# Autodesk Inventor assembly: 372.91.330
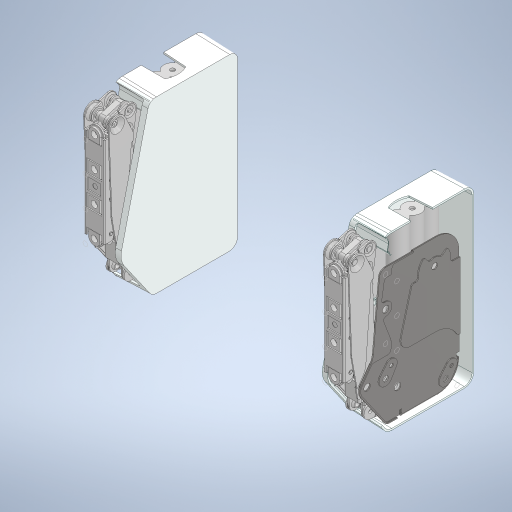
[picture p0: Inventor's stored thumbnail of the model, 512x512]
Saved by Autodesk Inventor 2024 (Build 280153000, 153)
## iProperties
RuleStatus: InUse
Created: 2019-11-19
Part Number: 372.91.330
Document SubType Name: Assembly
Designer: RokasM
Description: Hafele Free flap 3.15 107 deg mod.D
AfterDocOpen0: FrontOffset
Title: Hafele Free flap 3.15 107 deg mod.D
Revision Number: 1
## Documents named in this file (21)
- C:\W4INV 2024 Design\LIBRARY\Flap Fittings & Stays\Hafele Free flap 3.15 107 deg mod.D\Hafele_Free_flap_3.15_107_deg_mod.D.iam
- C:\W4INV 2024 Design\LIBRARY\Flap Fittings & Stays\Hafele Free flap 3.15 107 deg mod.D\Parts\372.91.410.ipt
- C:\W4INV 2024 Design\LIBRARY\Flap Fittings & Stays\Hafele Free flap 3.15 107 deg mod.D\Parts\372.91.410_1.ipt
- C:\W4INV 2024 Design\LIBRARY\Flap Fittings & Stays\Hafele Free flap 3.15 107 deg mod.D\Parts\372.91.410_2.ipt
- C:\W4INV 2024 Design\LIBRARY\Flap Fittings & Stays\Hafele Free flap 3.15 107 deg mod.D\Parts\372.91.410_3.ipt
- C:\W4INV 2024 Design\LIBRARY\Flap Fittings & Stays\Hafele Free flap 3.15 107 deg mod.D\Parts\372.91.410_4.ipt
- C:\W4INV 2024 Design\LIBRARY\Flap Fittings & Stays\Hafele Free flap 3.15 107 deg mod.D\Parts\372.91.410_5.ipt
- C:\W4INV 2024 Design\LIBRARY\Flap Fittings & Stays\Hafele Free flap 3.15 107 deg mod.D\Parts\372.91.410_6.ipt
- C:\W4INV 2024 Design\LIBRARY\Flap Fittings & Stays\Hafele Free flap 3.15 107 deg mod.D\Parts\372.91.410_7.ipt
- C:\W4INV 2024 Design\LIBRARY\Flap Fittings & Stays\Hafele Free flap 3.15 107 deg mod.D\Parts\372.91.433.ipt
- C:\W4INV 2024 Design\LIBRARY\Flap Fittings & Stays\Hafele Free flap 3.15 107 deg mod.D\Parts\372.91.410left.ipt
- C:\W4INV 2024 Design\LIBRARY\Flap Fittings & Stays\Hafele Free flap 3.15 107 deg mod.D\Parts\372.91.410_1left.ipt
- C:\W4INV 2024 Design\LIBRARY\Flap Fittings & Stays\Hafele Free flap 3.15 107 deg mod.D\Parts\372.91.410_2left.ipt
- C:\W4INV 2024 Design\LIBRARY\Flap Fittings & Stays\Hafele Free flap 3.15 107 deg mod.D\Parts\372.91.410_3left.ipt
- C:\W4INV 2024 Design\LIBRARY\Flap Fittings & Stays\Hafele Free flap 3.15 107 deg mod.D\Parts\372.91.410_4left.ipt
- C:\W4INV 2024 Design\LIBRARY\Flap Fittings & Stays\Hafele Free flap 3.15 107 deg mod.D\Parts\372.91.410_5left.ipt
- C:\W4INV 2024 Design\LIBRARY\Flap Fittings & Stays\Hafele Free flap 3.15 107 deg mod.D\Parts\372.91.410_6left.ipt
- C:\W4INV 2024 Design\LIBRARY\Flap Fittings & Stays\Hafele Free flap 3.15 107 deg mod.D\Parts\372.91.410_7left.ipt
- C:\W4INV 2024 Design\LIBRARY\Flap Fittings & Stays\Hafele Free flap 3.15 107 deg mod.D\Parts\372.91.433left.ipt
- C:\W4INV 2024 Design\LIBRARY\Flap Fittings & Stays\Hafele Free flap 3.15 107 deg mod.D\Parts\front_holes.ipt
- C:\Users\Public\Documents\Woodwork for Inventor\Textures\Black.png
## Components (20 placed, 19 different names)
1. cylinders:1 — Flush:4, Mate:4, Mate:5, Mate:6
2. door_plate:1 — Insert:5, Insert:6, Insert:7, Flush:18, Mate:20, Mate:21, Mate:22, Mate:23, Mate:27
3. upper_arm:1 — Insert:4, Insert:7, Mate:19
4. lower_arm:1 — Insert:3, Insert:6
5. swing_arm:1 — Insert:2, Insert:3
6. middle_arm:1 — Insert:1, Insert:5
7. outer_plate:1 — Flush:1, Flush:2, Flush:3, Mate:3, Flush:4, Mate:4, Mate:5, Angle:1, Flush:16, Flush:17
8. inner_plate:1 — Insert:1, Insert:2, Insert:4, Mate:1, Mate:2, Flush:2, Flush:3, Mate:3, Mate:6
9. cover:1 — Mate:1, Mate:2, Flush:1
10. cylinders_left:1 — Mate:10, Mate:11, Flush:9, Mate:12
11. door_plate_left:1 — Insert:8, Insert:9, Insert:11, Flush:18, Mate:19, Mate:20, Mate:24, Mate:25, Mate:26, Mate:28
12. upper_arm_left:1 — Insert:8, Insert:12
13. lower_arm_left:1 — Insert:9, Insert:10
14. swing_arm_left:1 — Insert:10, Insert:13
15. middle_arm_left:1 — Insert:11, Insert:14
16. outer_plate_left:1 — Mate:10, Mate:11, Flush:9, Mate:13, Flush:10, Flush:11, Flush:12, Flush:16, Flush:17
17. inner_plate_left:1 — Mate:12, Mate:13, Flush:10, Flush:11, Insert:12, Insert:13, Insert:14, Mate:14, Mate:15
18. cover_left:1 — Flush:12, Mate:14, Mate:15
19. front_holes:1 — Mate:21, Mate:22, Mate:23, Mate:27
20. front_holes:2 — Mate:24, Mate:25, Mate:26, Mate:28
## Relationships (48: Mate 22, Insert 14, Flush 11, Angle 1)
- Insert:1 (7.2 mm): middle_arm:1 ↔ inner_plate:1
- Insert:2 (2 mm): swing_arm:1 ↔ inner_plate:1
- Insert:3 (-0.55 mm): lower_arm:1 ↔ swing_arm:1
- Insert:4 (-0.3 mm): upper_arm:1 ↔ inner_plate:1
- Insert:5 (0.25 mm): door_plate:1 ↔ middle_arm:1
- Insert:6 (2.05 mm): door_plate:1 ↔ lower_arm:1
- Insert:7 (0.15 mm): door_plate:1 ↔ upper_arm:1
- Mate:1: inner_plate:1 ↔ cover:1
- Mate:2: inner_plate:1 ↔ cover:1
- Flush:1: outer_plate:1 ↔ cover:1
- Flush:2: outer_plate:1 ↔ inner_plate:1
- Flush:3: outer_plate:1 ↔ inner_plate:1
- Mate:3 (26.2 mm): outer_plate:1 ↔ inner_plate:1
- Flush:4 (-24.9 mm): cylinders:1 ↔ outer_plate:1
- Mate:4 (-14.3 mm): cylinders:1 ↔ outer_plate:1
- Mate:5 (-14.3 mm): cylinders:1 ↔ outer_plate:1
- Mate:6 (-19.92 mm): cylinders:1 ↔ inner_plate:1
- Angle:1 (0 deg): outer_plate:1
- Insert:8 (0.15 mm): door_plate_left:1 ↔ upper_arm_left:1
- Insert:9 (2.05 mm): door_plate_left:1 ↔ lower_arm_left:1
- Insert:10 (-0.55 mm): lower_arm_left:1 ↔ swing_arm_left:1
- Insert:11 (0.25 mm): door_plate_left:1 ↔ middle_arm_left:1
- Mate:10 (-14.3 mm): cylinders_left:1 ↔ outer_plate_left:1
- Mate:11 (-14.3 mm): cylinders_left:1 ↔ outer_plate_left:1
- Flush:9 (-24.9 mm): cylinders_left:1 ↔ outer_plate_left:1
- Mate:12 (-19.92 mm): cylinders_left:1 ↔ inner_plate_left:1
- Mate:13 (26.2 mm): outer_plate_left:1 ↔ inner_plate_left:1
- Flush:10: outer_plate_left:1 ↔ inner_plate_left:1
- Flush:11: outer_plate_left:1 ↔ inner_plate_left:1
- Insert:12 (-0.3 mm): upper_arm_left:1 ↔ inner_plate_left:1
- Insert:13 (2 mm): swing_arm_left:1 ↔ inner_plate_left:1
- Insert:14 (7.2 mm): middle_arm_left:1 ↔ inner_plate_left:1
- Flush:12: outer_plate_left:1 ↔ cover_left:1
- Mate:14: inner_plate_left:1 ↔ cover_left:1
- Mate:15: inner_plate_left:1 ↔ cover_left:1
- Flush:16: outer_plate:1 ↔ outer_plate_left:1
- Flush:17: outer_plate:1 ↔ outer_plate_left:1
- Flush:18: door_plate:1 ↔ door_plate_left:1
- Mate:19: upper_arm:1 ↔ door_plate_left:1
- Mate:20: door_plate:1 ↔ door_plate_left:1
- Mate:21 (-0.529 mm): door_plate:1 ↔ front_holes:1
- Mate:22 (7.377 mm): door_plate:1 ↔ front_holes:1
- Mate:23 (-6.5 mm): door_plate:1 ↔ front_holes:1
- Mate:24 (-0.529 mm): door_plate_left:1 ↔ front_holes:2
- Mate:25 (7.377 mm): door_plate_left:1 ↔ front_holes:2
- Mate:26 (-6.5 mm): door_plate_left:1 ↔ front_holes:2
- Mate:27 (-6.5 mm): door_plate:1 ↔ front_holes:1
- Mate:28 (-6.5 mm): door_plate_left:1 ↔ front_holes:2
## Named parameters: zero_offset = -2.529 mm, user_offset = 2 mm, front_offset = -0.529 mm
